# Autodesk Inventor assembly: Extruder Head
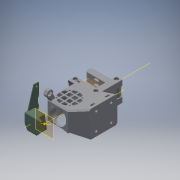
[picture p0: Inventor's stored thumbnail of the model, 180x180]
Saved by Autodesk Inventor 2018 (Build 220112000, 112)
## iProperties
Created: 2018-05-13
Part Number: Extruder Head
Document SubType Name: Assembly
Designer: Jasper
Author: Jasper
## Documents named in this file (14)
- C:\Users\Jasper\Downloads\git_WSL\MEME_MACHINE\CAD\Extruder\Extruder Head.iam
- C:\Users\Jasper\Downloads\git_WSL\MEME_MACHINE\CAD\Vitamins\Extruder.ipt
- C:\Users\Jasper\Downloads\git_WSL\MEME_MACHINE\CAD\Vitamins\NEMA17.ipt
- C:\Users\Jasper\Downloads\git_WSL\MEME_MACHINE\CAD\Vitamins\Hobbed Pulley.ipt
- C:\Users\Jasper\Downloads\git_WSL\MEME_MACHINE\CAD\Vitamins\625 Bearing.ipt
- C:\Users\Jasper\Downloads\git_WSL\MEME_MACHINE\CAD\Extruder\Extruder Body.ipt
- C:\Users\Jasper\Downloads\git_WSL\MEME_MACHINE\CAD\Vitamins\30mm Fan\30mm Fan.iam
- C:\Users\Jasper\Downloads\git_WSL\MEME_MACHINE\CAD\Extruder\Extruder Clamp.ipt
- C:\Users\Jasper\Downloads\git_WSL\MEME_MACHINE\CAD\Vitamins\50mm Blower Fan\Radial-Cooling-Fan-5015-DC12V.iam
- C:\Users\Jasper\Downloads\git_WSL\MEME_MACHINE\CAD\Extruder\Fan Shroud.ipt
- C:\Users\Jasper\Downloads\git_WSL\MEME_MACHINE\CAD\x-carriage-with-endstop-trigger.ipt
- D:\Jasper's Stuff\git_WSL\MEME_MACHINE\CAD\Vitamins\50mm Blower Fan\x-end-motor.ipt
- C:\Users\Jasper\Downloads\git_WSL\MEME_MACHINE\CAD\Extruder\Extruder Body Right.ipt
- C:\Users\Jasper\Downloads\git_WSL\MEME_MACHINE\CAD\Extruder\Extruder Body Left.ipt
## Components (13 placed, 13 different names)
1. Extruder:1 — Mate:2, Tangent:2, Angle:4, Tangent:3, Mate:7, Mate:8, Mate:10, Flush:5, Flush:7, Flush:8, Mate:22
2. NEMA17:1 — Mate:1, Angle:1, Flush:4, Angle:2, Mate:4, Angle:3, Angle:4, Tangent:3, Angle:5, Angle:7, Tangent:4, Mate:28, Mate:29
3. Hobbed Pulley:1 — Mate:1, Angle:1, Tangent:1, Mate:2, Angle:2
4. 625 Bearing:1 — Tangent:1, Tangent:2, Mate:3, Mate:13, Mate:14, Mate:15
5. Extruder Body:1 — Flush:4, Mate:12, Mate:16, Angle:9, Tangent:5, Mate:23, Angle:10, Angle:11
6. 30mm Fan:1 [sub-assembly] — Angle:8, Mate:11, Flush:5, Mate:12
7. Extruder Clamp:1 — Mate:13, Mate:15
8. Radial-Cooling-Fan-5015-DC12V:1 [sub-assembly] — Mate:16, Angle:9, Tangent:4, Tangent:5, Flush:6
9. Fan Shroud:1 — Flush:6, Mate:19, Flush:8, Mate:22
10. x-carriage-with-endstop-trigger:1 — Mate:23, Angle:10, Angle:12, Mate:24, Mate:25, Mate:26, Mate:27
11. x-end-motor:1 — Angle:11, Angle:12, Mate:24, Mate:25
12. Extruder Body Right — Mate:26, Mate:30, Flush:9
13. Extruder Body Left — Mate:27, Mate:28, Mate:29, Mate:30, Flush:9
## Relationships (50: Mate 28, Angle 11, Flush 6, Tangent 5)
- Mate:1: NEMA17:1 ↔ Hobbed Pulley:1
- Angle:1 (180 deg): NEMA17:1 ↔ Hobbed Pulley:1
- Tangent:1: Hobbed Pulley:1 ↔ 625 Bearing:1
- Flush:4: NEMA17:1 ↔ Extruder Body:1
- Mate:2: Extruder:1 ↔ Hobbed Pulley:1
- Tangent:2 (3 mm): Extruder:1 ↔ 625 Bearing:1
- Angle:2 (90 deg): NEMA17:1 ↔ Hobbed Pulley:1
- Mate:3: 625 Bearing:1
- Mate:4: NEMA17:1
- Mate:5
- Mate:6
- Angle:3 (0 deg): NEMA17:1
- Angle:4 (0 deg): Extruder:1 ↔ NEMA17:1
- Tangent:3 (5 mm): Extruder:1 ↔ NEMA17:1
- Mate:7: Extruder:1
- Angle:5 (0 deg): NEMA17:1
- Mate:8: Extruder:1
- Mate:10: Extruder:1
- Angle:7 (0 deg): NEMA17:1
- Angle:8 (0 deg): 30mm Fan:1
- Mate:11: 30mm Fan:1
- Flush:5: Extruder:1 ↔ 30mm Fan:1
- Mate:12: Extruder Body:1 ↔ 30mm Fan:1
- Mate:13: 625 Bearing:1 ↔ Extruder Clamp:1
- Mate:14: 625 Bearing:1
- Mate:15: 625 Bearing:1 ↔ Extruder Clamp:1
- Mate:16: Extruder Body:1 ↔ Radial-Cooling-Fan-5015-DC12V:1
- Angle:9 (0 deg): Extruder Body:1 ↔ Radial-Cooling-Fan-5015-DC12V:1
- Tangent:4 (-1 mm): NEMA17:1 ↔ Radial-Cooling-Fan-5015-DC12V:1
- Tangent:5 (1 mm): Extruder Body:1 ↔ Radial-Cooling-Fan-5015-DC12V:1
- Flush:6: Radial-Cooling-Fan-5015-DC12V:1 ↔ Fan Shroud:1
- Flush:7 (1.25 mm): Extruder:1
- Mate:17
- Mate:18
- Mate:19: Fan Shroud:1
- Mate:20
- Flush:8: Extruder:1 ↔ Fan Shroud:1
- Mate:22: Extruder:1 ↔ Fan Shroud:1
- Mate:23 (20 mm): Extruder Body:1 ↔ x-carriage-with-endstop-trigger:1
- Angle:10 (0 deg): Extruder Body:1 ↔ x-carriage-with-endstop-trigger:1
- Angle:11 (0 deg): Extruder Body:1 ↔ x-end-motor:1
- Angle:12 (180 deg): x-carriage-with-endstop-trigger:1 ↔ x-end-motor:1
- Mate:24: x-carriage-with-endstop-trigger:1 ↔ x-end-motor:1
- Mate:25: x-carriage-with-endstop-trigger:1 ↔ x-end-motor:1
- Mate:26: x-carriage-with-endstop-trigger:1 ↔ Extruder Body Right
- Mate:27: x-carriage-with-endstop-trigger:1 ↔ Extruder Body Left
- Mate:28: NEMA17:1 ↔ Extruder Body Left
- Mate:29: NEMA17:1 ↔ Extruder Body Left
- Mate:30: Extruder Body Right ↔ Extruder Body Left
- Flush:9: Extruder Body Right ↔ Extruder Body Left
